# Autodesk Inventor assembly: Mon-05_P1_Final_Deliverable_CAD
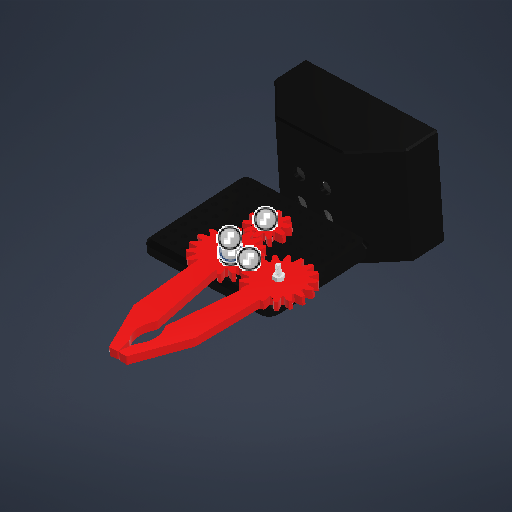
[picture p0: Inventor's stored thumbnail of the model, 512x512]
Saved by Autodesk Inventor 2026.1 (Build 301233000, 233)
## iProperties
Created: 2025-07-17
Part Number: Mon-05_P1_Final_Deliverable_CAD
Document SubType Name: Assembly
Designer: AdminForWorker
Title: End Effector Platform v38
Author: AdminForWorker
## Documents named in this file (13)
- C:\Users\charl\OneDrive - McMaster University\1P13\Design Studio\Mon-05_P1_Final_Deliverable_CAD.iam
- C:\Users\charl\OneDrive - McMaster University\1P13\Design Studio\End Effector Platform Models\N20 Mini Micro Metall Gear Motor DC 3-6-12V v1 v1.ipt
- C:\Users\charl\OneDrive - McMaster University\1P13\Design Studio\End Effector Platform Models\XC-430_idle v3.iam
- C:\Users\charl\OneDrive - McMaster University\1P13\Design Studio\End Effector Platform Models\End Effector Platform Base.ipt
- C:\Users\charl\OneDrive - McMaster University\1P13\Design Studio\End Effector Platform Models\Quanser QUARC EE Board.ipt
- C:\Users\charl\OneDrive - McMaster University\1P13\Design Studio\End Effector Platform Models\End Effector Platform.ipt
- C:\Users\charl\OneDrive - McMaster University\1P13\Design Studio\End Effector Platform Models\End Effector Platform Compartment Lid.ipt
- C:\Users\charl\OneDrive - McMaster University\1P13\Design Studio\End Effector Platform Models\Gripper Motor Cover.ipt
- C:\Users\charl\OneDrive - McMaster University\1P13\Design Studio\End Effector Platform Models\Fasteners\Steel M3x16 Pan Head Screw.ipt
- C:\Users\charl\OneDrive - McMaster University\1P13\Design Studio\End Effector Platform Models\Fasteners\Steel M3 Hex Nut.ipt
- C:\Users\charl\OneDrive - McMaster University\1P13\Design Studio\Left Arm.ipt
- C:\Users\charl\OneDrive - McMaster University\1P13\Design Studio\Right Arm.ipt
- C:\Users\charl\OneDrive - McMaster University\1P13\Design Studio\Driving Gear.ipt
## Components (14 placed, 10 different names)
1. N20 Mini Micro Metall Gear Motor DC 3-6-12V v1 v1:1 — Flush:3, Mate:8, Mate:9, Mate:10, Mate:11, Mate:12, Insert:10
2. XC-430_idle v3:1 [sub-assembly] — Mate:4, Mate:5, Mate:6
3. End Effector Platform Base:1 — Mate:1, Mate:2, Mate:3, Mate:4, Mate:5, Mate:6, Flush:1, Flush:2, Mate:7, Flush:3, Mate:8, Mate:9
4. Quanser QUARC EE Board:1 — Mate:1, Mate:2, Mate:3
5. End Effector Platform:1 — Mate:10, Mate:11, Mate:12, Mate:13, Flush:4, Flush:5, Insert:2, Insert:8, Insert:9, Mate:14, Mate:15, Angle:4, Angle:5, Angle:6, Angle:8
6. End Effector Platform Compartment Lid:1 — Flush:1, Flush:2, Mate:7
7. Gripper Motor Cover:1 — Mate:13, Flush:4, Flush:5
8. Steel M3x16 Pan Head Screw:1 — Mate:14, Mate:15, Angle:4
9. Steel M3x16 Pan Head Screw:2 — Insert:2, Angle:5
10. Steel M3 Hex Nut:1 — Mate:17, Angle:8, Angle:9
11. Steel M3 Hex Nut:2 — Mate:16, Angle:6, Angle:7
12. Spur Gear1:4 — Insert:8, Rotation:4, Angle:3, Mate:16, Angle:7
13. Spur Gear1:5 — Insert:9, Rotation:3, Rotation:4, Angle:2, Mate:17, Angle:9
14. Spur Gear1:6 — Insert:10, Rotation:3, Angle:1
## Relationships (37: Mate 17, Angle 9, Flush 5, Insert 4, RelateRotation 2)
- Mate:1: End Effector Platform Base:1 ↔ Quanser QUARC EE Board:1
- Mate:2: End Effector Platform Base:1 ↔ Quanser QUARC EE Board:1
- Mate:3: End Effector Platform Base:1 ↔ Quanser QUARC EE Board:1
- Mate:4: XC-430_idle v3:1 ↔ End Effector Platform Base:1
- Mate:5: XC-430_idle v3:1 ↔ End Effector Platform Base:1
- Mate:6: XC-430_idle v3:1 ↔ End Effector Platform Base:1
- Flush:1: End Effector Platform Base:1 ↔ End Effector Platform Compartment Lid:1
- Flush:2: End Effector Platform Base:1 ↔ End Effector Platform Compartment Lid:1
- Mate:7: End Effector Platform Base:1 ↔ End Effector Platform Compartment Lid:1
- Flush:3: N20 Mini Micro Metall Gear Motor DC 3-6-12V v1 v1:1 ↔ End Effector Platform Base:1
- Mate:8 (0.2 mm): N20 Mini Micro Metall Gear Motor DC 3-6-12V v1 v1:1 ↔ End Effector Platform Base:1
- Mate:9 (0.2 mm): N20 Mini Micro Metall Gear Motor DC 3-6-12V v1 v1:1 ↔ End Effector Platform Base:1
- Mate:10: N20 Mini Micro Metall Gear Motor DC 3-6-12V v1 v1:1 ↔ End Effector Platform:1
- Mate:11: N20 Mini Micro Metall Gear Motor DC 3-6-12V v1 v1:1 ↔ End Effector Platform:1
- Mate:12: N20 Mini Micro Metall Gear Motor DC 3-6-12V v1 v1:1 ↔ End Effector Platform:1
- Mate:13: End Effector Platform:1 ↔ Gripper Motor Cover:1
- Flush:4: End Effector Platform:1 ↔ Gripper Motor Cover:1
- Flush:5: End Effector Platform:1 ↔ Gripper Motor Cover:1
- Insert:2: End Effector Platform:1 ↔ Steel M3x16 Pan Head Screw:2
- Insert:8: End Effector Platform:1 ↔ Spur Gear1:4
- Insert:9: End Effector Platform:1 ↔ Spur Gear1:5
- Insert:10 (-8.3 mm): N20 Mini Micro Metall Gear Motor DC 3-6-12V v1 v1:1 ↔ Spur Gear1:6
- Rotation:3 [RelateRotation] (0.5882 ul): Spur Gear1:5 ↔ Spur Gear1:6
- Rotation:4 [RelateRotation] (1 ul): Spur Gear1:4 ↔ Spur Gear1:5
- Angle:1 (0 deg): Spur Gear1:6
- Angle:2 (-24.4 deg): Spur Gear1:5
- Angle:3 (0 deg): Spur Gear1:4
- Mate:14: End Effector Platform:1 ↔ Steel M3x16 Pan Head Screw:1
- Mate:15: End Effector Platform:1 ↔ Steel M3x16 Pan Head Screw:1
- Angle:4 (0 deg): End Effector Platform:1 ↔ Steel M3x16 Pan Head Screw:1
- Angle:5 (0 deg): End Effector Platform:1 ↔ Steel M3x16 Pan Head Screw:2
- Mate:16: Steel M3 Hex Nut:2 ↔ Spur Gear1:4
- Angle:6 (0 deg): End Effector Platform:1 ↔ Steel M3 Hex Nut:2
- Angle:7 (0 deg): Steel M3 Hex Nut:2 ↔ Spur Gear1:4
- Mate:17: Steel M3 Hex Nut:1 ↔ Spur Gear1:5
- Angle:8 (0 deg): End Effector Platform:1 ↔ Steel M3 Hex Nut:1
- Angle:9 (0 deg): Steel M3 Hex Nut:1 ↔ Spur Gear1:5
